# Autodesk Inventor assembly: ElectronicsBay
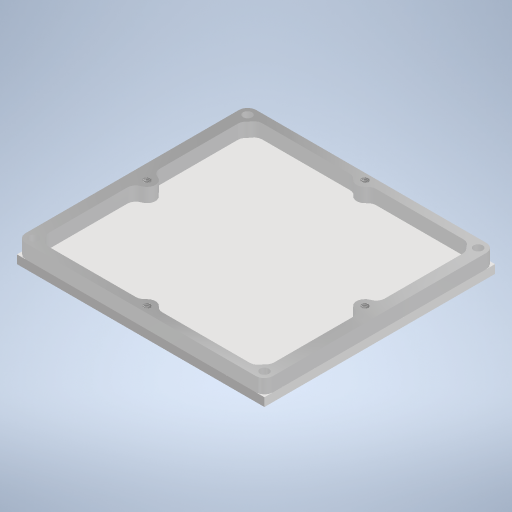
[picture p0: Inventor's stored thumbnail of the model, 512x512]
Saved by Autodesk Inventor 2023 (Build 270158000, 158)
## iProperties
Created: 2022-08-17
Part Number: ElectronicsBay
Document SubType Name: Assembly
Designer: Aditya Bansal
Author: Aditya Bansal
## Documents named in this file (3)
- C:\Users\Aditya Bansal\OneDrive - UNSW\Uni\BlueSat\rocketry-datasat\Structure\Electronics_Structure\ElectronicsBay.iam
- C:\Users\Aditya Bansal\OneDrive - UNSW\Uni\BlueSat\rocketry-datasat\Structure\Electronics_Structure\DummyPowerBoard.ipt
- C:\Users\Aditya Bansal\OneDrive - UNSW\Uni\BlueSat\rocketry-datasat\Structure\Electronics_Structure\ElectronicsBayMount.ipt
## Components (2 placed, 2 different names)
1. DummyPowerBoard:1 — Mate:1, Mate:2
2. ElectronicsBayMount:1 — Mate:1, Mate:2
## Relationships (2: Mate 2)
- Mate:1: DummyPowerBoard:1 ↔ ElectronicsBayMount:1
- Mate:2: DummyPowerBoard:1 ↔ ElectronicsBayMount:1
